# Autodesk Inventor assembly: case
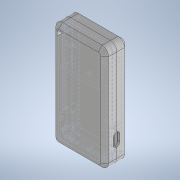
[picture p0: Inventor's stored thumbnail of the model, 180x180]
Saved by Autodesk Inventor 2020 (Build 240168000, 168)
## iProperties
Created: 2020-03-15
Part Number: case
Document SubType Name: Assembly
Designer: erwin
Author: erwin
## Documents named in this file (7)
- C:\Users\erwin\Documents\GitHub\pidflight-lap-firmware\case\case.iam
- C:\Users\erwin\Documents\GitHub\pidflight-lap-firmware\case\lipo.ipt
- C:\Users\erwin\Documents\GitHub\pidflight-lap-firmware\case\esp32_t8.ipt
- C:\Users\erwin\Documents\GitHub\pidflight-lap-firmware\case\rx5808.ipt
- C:\Users\erwin\Documents\GitHub\pidflight-lap-firmware\case\switch.ipt
- C:\Users\erwin\Documents\GitHub\pidflight-lap-firmware\case\case_up.ipt
- C:\Users\erwin\Documents\GitHub\pidflight-lap-firmware\case\case_down.ipt
## Components (6 placed, 6 different names)
1. lipo:1
2. esp32_t8:1 — Flush:4, Flush:5
3. rx5808:1
4. switch:1 — Flush:4, Flush:5
5. case_up:1
6. case_down:1
## Relationships (2: Flush 2)
- Flush:4: esp32_t8:1 ↔ switch:1
- Flush:5: esp32_t8:1 ↔ switch:1
